# Autodesk Inventor assembly: elbowassembly
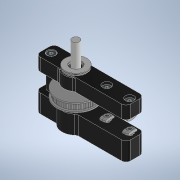
[picture p0: Inventor's stored thumbnail of the model, 180x180]
Saved by Autodesk Inventor 2022 (Build 260153000, 153)
## iProperties
Created: 2022-02-22
Part Number: elbowassembly
Document SubType Name: Assembly
Designer: JK
Author: JK
## Documents named in this file (14)
- C:\Users\JK\Documents\Inventor\ScaraNema\SCARA-3DP\Parts\Arm\Elbow assembly.iam
- C:\Users\JK\Documents\Inventor\ScaraNema\SCARA-3DP\Parts\Common components\GT260T.ipt
- C:\Users\JK\Documents\Inventor\ScaraNema\SCARA-3DP\Parts\Arm\Top pulley support.ipt
- C:\Users\JK\Documents\Inventor\ScaraNema\SCARA-3DP\Parts\Arm\Bottom pulley support.ipt
- C:\Users\JK\Documents\Inventor\ScaraNema\SCARA-3DP\Parts\Arm\8x80 mm axis.ipt
- C:\Users\JK\Documents\Inventor\ScaraNema\SCARA-3DP\Parts\Fasteners\M5 Hex nut.ipt
- C:\Users\JK\Documents\Inventor\ScaraNema\SCARA-3DP\Parts\Fasteners\M5x15 Flat head bolt.ipt
- C:\Users\JK\Documents\Inventor\ScaraNema\SCARA-3DP\Parts\Fasteners\M5 T-Nut Drop-in 20x20.ipt
- C:\Users\JK\Documents\Inventor\ScaraNema\SCARA-3DP\Parts\Arm\5909K31_Needle-Roller Thrust Bearing.ipt
- C:\Users\JK\Documents\Inventor\ScaraNema\SCARA-3DP\Parts\Arm\5909K44_0.032 Thick Washer for 1 2 Shaft Diameter Needle-Roller Thrust Bearing.ipt
- C:\Users\JK\Documents\Inventor\ScaraNema\SCARA-3DP\Parts\Common components\688-2RS.ipt
- C:\Users\JK\Documents\Inventor\ScaraNema\SCARA-3DP\Parts\Arm\Pulley support separator.ipt
- C:\Users\JK\Documents\Inventor\ScaraNema\SCARA-3DP\Parts\Fasteners\M5x20 Flat head bolt.ipt
- C:\Users\JK\Documents\Inventor\ScaraNema\SCARA-3DP\Parts\Fasteners\M5x50 Flat head bolt.ipt
## Components (20 placed, 13 different names)
1. GT260T:1 — Coincidencia:63, Coincidencia:64
2. Bottom pulley support:1 — Coincidencia:29, Coincidencia:31, Ángulo:1, Nivelación:2, Coincidencia:45, Nivelación:6, Coincidencia:60, Coincidencia:65, Coincidencia:67, Coincidencia:68, Coincidencia:69, Coincidencia:72
3. Top pulley support:1 — Coincidencia:29, Coincidencia:33, Coincidencia:34, Coincidencia:35, Coincidencia:36, Nivelación:2, Ángulo:3, Coincidencia:39, Coincidencia:46, Coincidencia:51, Coincidencia:54, Coincidencia:55, Coincidencia:58, Coincidencia:64, Coincidencia:66
4. 8x80 mm axis:1 — Coincidencia:36, Nivelación:6, Coincidencia:50, Coincidencia:52, Coincidencia:53, Coincidencia:56, Coincidencia:63
5. M5 Hex nut:2 — Coincidencia:31, Ángulo:1, Coincidencia:72
6. M5x15 Flat head bolt:1 — Coincidencia:34, Nivelación:1, Coincidencia:35, Coincidencia:37
7. M5x15 Flat head bolt:2 — Coincidencia:33, Nivelación:1, Coincidencia:38
8. M5 T-Nut Drop-in 20x20:1 — Coincidencia:38, Ángulo:2, Nivelación:3, Coincidencia:39, Ángulo:5
9. M5 T-Nut Drop-in 20x20:2 — Coincidencia:37, Ángulo:2, Ángulo:3, Nivelación:3
10. M5 T-Nut Drop-in 20x20:3 — Nivelación:5, Ángulo:4, Ángulo:5, Coincidencia:45, Coincidencia:71
11. M5 T-Nut Drop-in 20x20:4 — Nivelación:5, Ángulo:4, Coincidencia:70
12. M5x50 Flat head bolt:1 — Coincidencia:46, Coincidencia:58, Coincidencia:59
13. 5909K31_Needle-Roller Thrust Bearing:1 — Coincidencia:52, Tangente:1, Tangente:2
14. 5909K44_0.032 Thick Washer for 1 2 Shaft Diameter Needle-Roller Thrust Bearing:1 — Coincidencia:50, Coincidencia:51, Tangente:1
15. 5909K44_0.032 Thick Washer for 1 2 Shaft Diameter Needle-Roller Thrust Bearing:2 — Tangente:2, Coincidencia:53
16. 688-2RS:1 — Coincidencia:54, Coincidencia:55
17. 688-2RS:2 — Coincidencia:56, Coincidencia:65
18. Pulley support separator:1 — Coincidencia:59, Coincidencia:60, Coincidencia:66
19. M5x20 Flat head bolt:1 — Coincidencia:67, Nivelación:7, Coincidencia:69, Coincidencia:71
20. M5x20 Flat head bolt:2 — Coincidencia:68, Nivelación:7, Coincidencia:70
## Relationships (44: Mate 31, Flush 6, Angle 5, Tangent 2)
- Coincidencia:29 [Mate]: Bottom pulley support:1 ↔ Top pulley support:1
- Coincidencia:31 [Mate]: Bottom pulley support:1 ↔ M5 Hex nut:2
- Ángulo:1 [Angle] (0 deg): Bottom pulley support:1 ↔ M5 Hex nut:2
- Coincidencia:33 [Mate]: Top pulley support:1 ↔ M5x15 Flat head bolt:2
- Coincidencia:34 [Mate]: Top pulley support:1 ↔ M5x15 Flat head bolt:1
- Nivelación:1 [Flush]: M5x15 Flat head bolt:1 ↔ M5x15 Flat head bolt:2
- Coincidencia:35 [Mate]: Top pulley support:1 ↔ M5x15 Flat head bolt:1
- Coincidencia:36 [Mate]: Top pulley support:1 ↔ 8x80 mm axis:1
- Nivelación:2 [Flush]: Bottom pulley support:1 ↔ Top pulley support:1
- Coincidencia:37 [Mate]: M5x15 Flat head bolt:1 ↔ M5 T-Nut Drop-in 20x20:2
- Coincidencia:38 [Mate]: M5x15 Flat head bolt:2 ↔ M5 T-Nut Drop-in 20x20:1
- Ángulo:2 [Angle] (0 deg): M5 T-Nut Drop-in 20x20:1 ↔ M5 T-Nut Drop-in 20x20:2
- Ángulo:3 [Angle] (90 deg): Top pulley support:1 ↔ M5 T-Nut Drop-in 20x20:2
- Nivelación:3 [Flush]: M5 T-Nut Drop-in 20x20:1 ↔ M5 T-Nut Drop-in 20x20:2
- Coincidencia:39 [Mate] (0.6 mm): Top pulley support:1 ↔ M5 T-Nut Drop-in 20x20:1
- Nivelación:5 [Flush]: M5 T-Nut Drop-in 20x20:3 ↔ M5 T-Nut Drop-in 20x20:4
- Ángulo:4 [Angle] (0 deg): M5 T-Nut Drop-in 20x20:3 ↔ M5 T-Nut Drop-in 20x20:4
- Ángulo:5 [Angle] (0 deg): M5 T-Nut Drop-in 20x20:1 ↔ M5 T-Nut Drop-in 20x20:3
- Coincidencia:45 [Mate] (0.6 mm): Bottom pulley support:1 ↔ M5 T-Nut Drop-in 20x20:3
- Nivelación:6 [Flush]: Bottom pulley support:1 ↔ 8x80 mm axis:1
- Coincidencia:46 [Mate]: Top pulley support:1 ↔ M5x50 Flat head bolt:1
- Coincidencia:50 [Mate]: 8x80 mm axis:1 ↔ 5909K44_0.032 Thick Washer for 1 2 Shaft Diameter Needle-Roller Thrust Bearing:1
- Coincidencia:51 [Mate]: Top pulley support:1 ↔ 5909K44_0.032 Thick Washer for 1 2 Shaft Diameter Needle-Roller Thrust Bearing:1
- Coincidencia:52 [Mate]: 8x80 mm axis:1 ↔ 5909K31_Needle-Roller Thrust Bearing:1
- Tangente:1: 5909K31_Needle-Roller Thrust Bearing:1 ↔ 5909K44_0.032 Thick Washer for 1 2 Shaft Diameter Needle-Roller Thrust Bearing:1
- Tangente:2: 5909K31_Needle-Roller Thrust Bearing:1 ↔ 5909K44_0.032 Thick Washer for 1 2 Shaft Diameter Needle-Roller Thrust Bearing:2
- Coincidencia:53 [Mate]: 8x80 mm axis:1 ↔ 5909K44_0.032 Thick Washer for 1 2 Shaft Diameter Needle-Roller Thrust Bearing:2
- Coincidencia:54 [Mate]: Top pulley support:1 ↔ 688-2RS:1
- Coincidencia:55 [Mate]: Top pulley support:1 ↔ 688-2RS:1
- Coincidencia:56 [Mate]: 8x80 mm axis:1 ↔ 688-2RS:2
- Coincidencia:58 [Mate]: Top pulley support:1 ↔ M5x50 Flat head bolt:1
- Coincidencia:59 [Mate]: M5x50 Flat head bolt:1 ↔ Pulley support separator:1
- Coincidencia:60 [Mate]: Bottom pulley support:1 ↔ Pulley support separator:1
- Coincidencia:63 [Mate]: GT260T:1 ↔ 8x80 mm axis:1
- Coincidencia:64 [Mate] (5 mm): GT260T:1 ↔ Top pulley support:1
- Coincidencia:65 [Mate]: Bottom pulley support:1 ↔ 688-2RS:2
- Coincidencia:66 [Mate]: Top pulley support:1 ↔ Pulley support separator:1
- Coincidencia:67 [Mate]: Bottom pulley support:1 ↔ M5x20 Flat head bolt:1
- Coincidencia:68 [Mate]: Bottom pulley support:1 ↔ M5x20 Flat head bolt:2
- Nivelación:7 [Flush]: M5x20 Flat head bolt:1 ↔ M5x20 Flat head bolt:2
- Coincidencia:69 [Mate]: Bottom pulley support:1 ↔ M5x20 Flat head bolt:1
- Coincidencia:70 [Mate]: M5 T-Nut Drop-in 20x20:4 ↔ M5x20 Flat head bolt:2
- Coincidencia:71 [Mate]: M5 T-Nut Drop-in 20x20:3 ↔ M5x20 Flat head bolt:1
- Coincidencia:72 [Mate]: Bottom pulley support:1 ↔ M5 Hex nut:2
